# Autodesk Inventor assembly: OktagonElektronik_Stage1
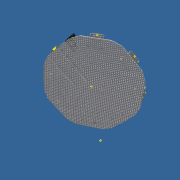
[picture p0: Inventor's stored thumbnail of the model, 180x180]
Saved by Autodesk Inventor 2018 (Build 220112000, 112)
## iProperties
Company: Fraunhofer ILT
Created: 2018-10-31
Part Number: OktagonElektronik_Stage1
Material: geeigneten Werkstoff auswählen !
Document SubType Name: Assembly
Designer: N.Grubert
Title: =Description
Author: N.Grubert
## Documents named in this file (7)
- C:\Users\knabe\Documents\Nicole\Uni\COSIMA\CAD\Oktokommander\OktagonElektronik_Stage1.iam
- C:\Users\knabe\Documents\Nicole\Uni\COSIMA\CAD\Oktokommander\ARDUINO MICRO.iam
- C:\Users\knabe\Documents\Nicole\Uni\COSIMA\CAD\Oktokommander\Polygonplatine.ipt
- C:\Users\knabe\Documents\Nicole\Uni\COSIMA\CAD\Oktokommander\USB_female.ipt
- C:\Users\knabe\Documents\Nicole\Uni\COSIMA\CAD\Oktokommander\16Bit I2C ADC+PGA - ADS1115.iam
- C:\Users\knabe\Documents\Nicole\Uni\COSIMA\CAD\Oktokommander\Adafruit.ipt
- C:\Users\knabe\Documents\Nicole\Uni\COSIMA\CAD\Oktokommander\2.1mm_DC_Power_Socket.ipt
## Components (12 placed, 6 different names)
1. ARDUINO MICRO:1 [sub-assembly] — Fluchtend:1, Passend:18, Fluchtend:18, Fluchtend:20, Winkel:5
2. Polygonplatine:1 — Passend:1, Passend:2, Passend:3, Passend:4, Passend:5, Passend:6, Passend:7, Fluchtend:1, Winkel:4, Fluchtend:2, Fluchtend:3, Fluchtend:7, Fluchtend:8, Fluchtend:9, Fluchtend:10, Fluchtend:11, Fluchtend:12, Fluchtend:13, Passend:18, Fluchtend:18, Passend:20, Fluchtend:19
3. USB_female:1 — Passend:2, Winkel:1, Fluchtend:5, Fluchtend:10
4. USB_female:2 — Passend:4, Winkel:4, Fluchtend:13
5. USB_female:3 — Passend:1, Winkel:2, Fluchtend:6, Fluchtend:7
6. USB_female:4 — Passend:3, Winkel:3, Fluchtend:3, Fluchtend:4
7. USB_female:5 — Passend:6, Winkel:3, Fluchtend:2, Fluchtend:4, Fluchtend:12
8. USB_female:6 — Passend:7, Winkel:2, Fluchtend:6, Fluchtend:8
9. USB_female:7 — Passend:5, Winkel:1, Fluchtend:5, Fluchtend:9, Fluchtend:11
10. 16Bit I2C ADC+PGA - ADS1115:1 [sub-assembly] — Fluchtend:20, Winkel:5, Fluchtend:21, Winkel:6, Fluchtend:22, Passend:21
11. Adafruit:1 — Fluchtend:21, Winkel:6, Fluchtend:22, Passend:21
12. 2.1mm_DC_Power_Socket:1 — Passend:20, Fluchtend:19
## Relationships (34: Flush 18, Mate 10, Angle 6)
- Passend:1 [Mate]: Polygonplatine:1 ↔ USB_female:3
- Passend:2 [Mate]: Polygonplatine:1 ↔ USB_female:1
- Passend:3 [Mate]: Polygonplatine:1 ↔ USB_female:4
- Passend:4 [Mate]: Polygonplatine:1 ↔ USB_female:2
- Passend:5 [Mate]: Polygonplatine:1 ↔ USB_female:7
- Passend:6 [Mate]: Polygonplatine:1 ↔ USB_female:5
- Passend:7 [Mate]: Polygonplatine:1 ↔ USB_female:6
- Fluchtend:1 [Flush]: ARDUINO MICRO:1 ↔ Polygonplatine:1
- Winkel:1 [Angle] (180 deg): USB_female:1 ↔ USB_female:7
- Winkel:2 [Angle] (180 deg): USB_female:3 ↔ USB_female:6
- Winkel:3 [Angle] (180 deg): USB_female:4 ↔ USB_female:5
- Winkel:4 [Angle] (180 deg): Polygonplatine:1 ↔ USB_female:2
- Fluchtend:2 [Flush]: Polygonplatine:1 ↔ USB_female:5
- Fluchtend:3 [Flush]: Polygonplatine:1 ↔ USB_female:4
- Fluchtend:4 [Flush]: USB_female:4 ↔ USB_female:5
- Fluchtend:5 [Flush]: USB_female:1 ↔ USB_female:7
- Fluchtend:6 [Flush]: USB_female:3 ↔ USB_female:6
- Fluchtend:7 [Flush]: Polygonplatine:1 ↔ USB_female:3
- Fluchtend:8 [Flush]: Polygonplatine:1 ↔ USB_female:6
- Fluchtend:9 [Flush]: Polygonplatine:1 ↔ USB_female:7
- Fluchtend:10 [Flush]: Polygonplatine:1 ↔ USB_female:1
- Fluchtend:11 [Flush]: Polygonplatine:1 ↔ USB_female:7
- Fluchtend:12 [Flush]: Polygonplatine:1 ↔ USB_female:5
- Fluchtend:13 [Flush]: Polygonplatine:1 ↔ USB_female:2
- Passend:18 [Mate]: ARDUINO MICRO:1 ↔ Polygonplatine:1
- Fluchtend:18 [Flush]: ARDUINO MICRO:1 ↔ Polygonplatine:1
- Passend:20 [Mate]: Polygonplatine:1 ↔ 2.1mm_DC_Power_Socket:1
- Fluchtend:19 [Flush]: Polygonplatine:1 ↔ 2.1mm_DC_Power_Socket:1
- Fluchtend:20 [Flush]: ARDUINO MICRO:1 ↔ 16Bit I2C ADC+PGA - ADS1115:1
- Winkel:5 [Angle] (90 deg): ARDUINO MICRO:1 ↔ 16Bit I2C ADC+PGA - ADS1115:1
- Fluchtend:21 [Flush]: 16Bit I2C ADC+PGA - ADS1115:1 ↔ Adafruit:1
- Winkel:6 [Angle] (90 deg): 16Bit I2C ADC+PGA - ADS1115:1 ↔ Adafruit:1
- Fluchtend:22 [Flush]: 16Bit I2C ADC+PGA - ADS1115:1 ↔ Adafruit:1
- Passend:21 [Mate] (5 mm): 16Bit I2C ADC+PGA - ADS1115:1 ↔ Adafruit:1
